# Autodesk Inventor assembly: Montagem1
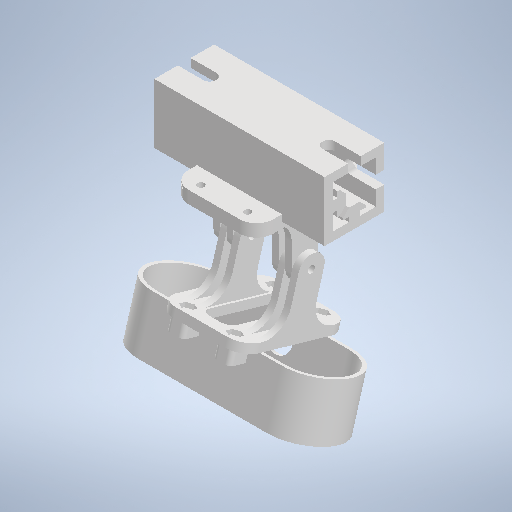
[picture p0: Inventor's stored thumbnail of the model, 512x512]
Saved by Autodesk Inventor 2025 (Build 290162000, 162)
## iProperties
Created: 2024-08-25
Part Number: Montagem1
Document SubType Name: Assembly
Designer: dvccs
Author: dvccs
## Documents named in this file (4)
- C:\Users\dvccs\Documents\Montagem1.iam
- C:\Users\dvccs\Desktop\projeto_prototipagem_CME\cameraSlider2.ipt
- C:\Users\dvccs\Desktop\projeto_prototipagem_CME\encaixeDuplo2.ipt
- C:\Users\dvccs\Desktop\projeto_prototipagem_CME\suporteBright2k.ipt
## Components (4 placed, 3 different names)
1. cameraSlider2:1 — Coincidente:1, Coincidente:2
2. encaixeDuplo2:1 — Coincidente:3, Coincidente:4, Coincidente:5, Coincidente:6, Coincidente:7
3. suporteBright2k:1 — Coincidente:5, Coincidente:6, Coincidente:7
4. encaixeDuplo2:2 — Coincidente:1, Coincidente:2, Coincidente:3, Coincidente:4
## Relationships (7: Mate 7)
- Coincidente:1 [Mate]: cameraSlider2:1 ↔ encaixeDuplo2:2
- Coincidente:2 [Mate]: cameraSlider2:1 ↔ encaixeDuplo2:2
- Coincidente:3 [Mate]: encaixeDuplo2:1 ↔ encaixeDuplo2:2
- Coincidente:4 [Mate]: encaixeDuplo2:1 ↔ encaixeDuplo2:2
- Coincidente:5 [Mate]: encaixeDuplo2:1 ↔ suporteBright2k:1
- Coincidente:6 [Mate]: encaixeDuplo2:1 ↔ suporteBright2k:1
- Coincidente:7 [Mate]: encaixeDuplo2:1 ↔ suporteBright2k:1
